# Autodesk Inventor assembly: VersaPlanetary Two Stage 775 Ratchet
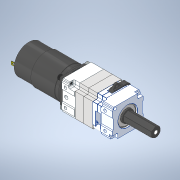
[picture p0: Inventor's stored thumbnail of the model, 180x180]
Saved by Autodesk Inventor 2020 (Build 240168000, 168)
## iProperties
Created: 2020-01-30
Part Number: VersaPlanetary Two Stage 775 Ratchet
Document SubType Name: Assembly
Designer: aidan
Author: aidan
## Documents named in this file (15)
- C:\Users\aidan\Desktop\T3 Robotics\CAD\Generic and Stock\VersaPlanetary Parts\VersaPlanetary Two Stage 775 Ratchet.iam
- C:\Users\aidan\Desktop\T3 Robotics\CAD\Generic and Stock\775 Pro.ipt
- C:\Users\aidan\Desktop\T3 Robotics\CAD\STEP Files\775_Series_Motor_Mounting_Plate.ipt
- C:\Users\aidan\Desktop\T3 Robotics\CAD\Generic and Stock\VersaPlanetary Parts\VersaPlanertary Mounting Block.ipt
- C:\Users\aidan\Desktop\T3 Robotics\CAD\Generic and Stock\VersaPlanetary Parts\VersaPlanetary Coupler.ipt
- C:\Users\aidan\Desktop\T3 Robotics\CAD\Generic and Stock\VersaPlanetary Parts\VersaPlanetary Motor Screw.ipt
- C:\Users\aidan\Desktop\T3 Robotics\CAD\Generic and Stock\VersaPlanetary Parts\VersaPlanetary Mounting Screw.ipt
- C:\Users\aidan\Desktop\T3 Robotics\CAD\Generic and Stock\VersaPlanetary Parts\VersaPlanetary Ring Gear.ipt
- C:\Users\aidan\Desktop\T3 Robotics\CAD\Generic and Stock\VersaPlanetary Parts\VersaPlanetary Long Screw.ipt
- C:\Users\aidan\Desktop\T3 Robotics\CAD\Generic and Stock\VersaPlanetary Parts\VersaPlanetary 0.500 Output.ipt
- C:\Users\aidan\Desktop\T3 Robotics\CAD\Generic and Stock\VersaPlanetary Parts\Ratchet Set Pin.ipt
- C:\Users\aidan\Desktop\T3 Robotics\CAD\Generic and Stock\VersaPlanetary Parts\Ratchet Set Ratchet.ipt
- C:\Users\aidan\Desktop\T3 Robotics\CAD\Generic and Stock\VersaPlanetary Parts\Ratchet Set Spacer.ipt
- C:\Users\aidan\Desktop\T3 Robotics\CAD\Generic and Stock\VersaPlanetary Parts\VersaPlanetary Ratchet Plate.iam
- C:\Users\aidan\Desktop\T3 Robotics\CAD\Generic and Stock\VersaPlanetary Parts\VersaPlanetary Ratchet Plate 2.ipt
## Components (19 placed, 14 different names)
1. 775 Pro:1 — Mate:9, Mate:10, Mate:15, Flush:7, Mate:16, Mate:22
2. 775_Series_Motor_Mounting_Plate:1 — Mate:6, Mate:7, Mate:8, Mate:10, Mate:13, Mate:19, Flush:9
3. VersaPlanertary Mounting Block:1 — Flush:2, Mate:2, Mate:3, Mate:19, Mate:20, Mate:21, Mate:22, Flush:9, Mate:23, Mate:24, Mate:25
4. VersaPlanetary Coupler:1 — Mate:15, Flush:7
5. VersaPlanetary Motor Screw:1 — Mate:6, Flush:5, Mate:8, Mate:16
6. VersaPlanetary Motor Screw:2 — Mate:7, Flush:5, Mate:9
7. VersaPlanetary Mounting Screw:1 — Flush:6, Mate:21
8. VersaPlanetary Mounting Screw:2 — Flush:6, Mate:13, Mate:20
9. VersaPlanetary Ring Gear:1 — Flush:1, Flush:2, Flush:4, Mate:1, Mate:2, Mate:3
10. VersaPlanetary Ring Gear:2 — Flush:1, Flush:3, Flush:4, Mate:1, Mate:5, Mate:34, Mate:38
11. VersaPlanetary Long Screw:1 — Flush:8, Mate:25
12. VersaPlanetary Long Screw:2 — Flush:8, Mate:23, Mate:24, Mate:39
13. VersaPlanetary 0.500 Output:1 — Flush:3, Mate:5, Mate:40, Mate:41, Angle:1
14. Ratchet Set Ratchet:1 — Mate:33, Mate:35, Mate:42
15. Ratchet Set Spacer:1 — Mate:28, Mate:29, Flush:10, Mate:33, Mate:39
16. VersaPlanetary Ratchet Plate:1 [sub-assembly] — Mate:26, Mate:27, Mate:29, Flush:10, Mate:31, Flush:11, Mate:34, Mate:35, Mate:36, Mate:41
17. VersaPlanetary Ratchet Plate 2:1 — Mate:26, Mate:27, Mate:28, Mate:30, Mate:38
18. Ratchet Set Spacer:2 — Mate:30, Mate:31, Flush:11
19. Ratchet Set Pin:1 — Mate:36, Mate:40
## Relationships (46: Mate 34, Flush 11, Angle 1)
- Flush:1: VersaPlanetary Ring Gear:1 ↔ VersaPlanetary Ring Gear:2
- Flush:2: VersaPlanertary Mounting Block:1 ↔ VersaPlanetary Ring Gear:1
- Flush:3: VersaPlanetary Ring Gear:2 ↔ VersaPlanetary 0.500 Output:1
- Flush:4: VersaPlanetary Ring Gear:1 ↔ VersaPlanetary Ring Gear:2
- Mate:1: VersaPlanetary Ring Gear:1 ↔ VersaPlanetary Ring Gear:2
- Mate:2: VersaPlanertary Mounting Block:1 ↔ VersaPlanetary Ring Gear:1
- Mate:3: VersaPlanertary Mounting Block:1 ↔ VersaPlanetary Ring Gear:1
- Mate:5: VersaPlanetary Ring Gear:2 ↔ VersaPlanetary 0.500 Output:1
- Mate:6: 775_Series_Motor_Mounting_Plate:1 ↔ VersaPlanetary Motor Screw:1
- Mate:7: 775_Series_Motor_Mounting_Plate:1 ↔ VersaPlanetary Motor Screw:2
- Flush:5: VersaPlanetary Motor Screw:1 ↔ VersaPlanetary Motor Screw:2
- Mate:8: 775_Series_Motor_Mounting_Plate:1 ↔ VersaPlanetary Motor Screw:1
- Mate:9: 775 Pro:1 ↔ VersaPlanetary Motor Screw:2
- Mate:10: 775 Pro:1 ↔ 775_Series_Motor_Mounting_Plate:1
- Flush:6: VersaPlanetary Mounting Screw:1 ↔ VersaPlanetary Mounting Screw:2
- Mate:13: 775_Series_Motor_Mounting_Plate:1 ↔ VersaPlanetary Mounting Screw:2
- Mate:15: 775 Pro:1 ↔ VersaPlanetary Coupler:1
- Flush:7 (5.334 mm): 775 Pro:1 ↔ VersaPlanetary Coupler:1
- Mate:16: 775 Pro:1 ↔ VersaPlanetary Motor Screw:1
- Mate:19: 775_Series_Motor_Mounting_Plate:1 ↔ VersaPlanertary Mounting Block:1
- Flush:8: VersaPlanetary Long Screw:1 ↔ VersaPlanetary Long Screw:2
- Mate:20: VersaPlanertary Mounting Block:1 ↔ VersaPlanetary Mounting Screw:2
- Mate:21: VersaPlanertary Mounting Block:1 ↔ VersaPlanetary Mounting Screw:1
- Mate:22: 775 Pro:1 ↔ VersaPlanertary Mounting Block:1
- Flush:9: 775_Series_Motor_Mounting_Plate:1 ↔ VersaPlanertary Mounting Block:1
- Mate:23: VersaPlanertary Mounting Block:1 ↔ VersaPlanetary Long Screw:2
- Mate:24: VersaPlanertary Mounting Block:1 ↔ VersaPlanetary Long Screw:2
- Mate:25: VersaPlanertary Mounting Block:1 ↔ VersaPlanetary Long Screw:1
- Mate:26: VersaPlanetary Ratchet Plate:1 ↔ VersaPlanetary Ratchet Plate 2:1
- Mate:27: VersaPlanetary Ratchet Plate:1 ↔ VersaPlanetary Ratchet Plate 2:1
- Mate:28: Ratchet Set Spacer:1 ↔ VersaPlanetary Ratchet Plate 2:1
- Mate:29: Ratchet Set Spacer:1 ↔ VersaPlanetary Ratchet Plate:1
- Flush:10: Ratchet Set Spacer:1 ↔ VersaPlanetary Ratchet Plate:1
- Mate:30: VersaPlanetary Ratchet Plate 2:1 ↔ Ratchet Set Spacer:2
- Mate:31: VersaPlanetary Ratchet Plate:1 ↔ Ratchet Set Spacer:2
- Flush:11: VersaPlanetary Ratchet Plate:1 ↔ Ratchet Set Spacer:2
- Mate:33: Ratchet Set Ratchet:1 ↔ Ratchet Set Spacer:1
- Mate:34: VersaPlanetary Ring Gear:2 ↔ VersaPlanetary Ratchet Plate:1
- Mate:35: Ratchet Set Ratchet:1 ↔ VersaPlanetary Ratchet Plate:1
- Mate:36: VersaPlanetary Ratchet Plate:1 ↔ Ratchet Set Pin:1
- Mate:38: VersaPlanetary Ring Gear:2 ↔ VersaPlanetary Ratchet Plate 2:1
- Mate:39: VersaPlanetary Long Screw:2 ↔ Ratchet Set Spacer:1
- Mate:40: VersaPlanetary 0.500 Output:1 ↔ Ratchet Set Pin:1
- Mate:41: VersaPlanetary 0.500 Output:1 ↔ VersaPlanetary Ratchet Plate:1
- Mate:42: Ratchet Set Ratchet:1
- Angle:1 (0 deg): VersaPlanetary 0.500 Output:1
